# Autodesk Inventor assembly: MotorJaguarBoard
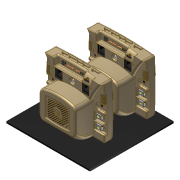
[picture p0: Inventor's stored thumbnail of the model, 180x180]
Saved by Autodesk Inventor 2012 (Build 160160000, 160)
## iProperties
Created: 2012-01-21
Part Number: MotorJaguarBoard
Document SubType Name: Assembly
Designer: JesseK
Author: JesseK
## Documents named in this file (3)
- Z:\UserData\Documents\Inventor\team1885frc\Robot2012\Electronics Board\MotorJaguarBoard.iam
- Z:\UserData\Documents\Inventor\team1885frc\Robot2012\Electronics Board\MotorJaguarBoard.ipt
- Z:\UserData\Documents\Inventor\team1885frc\Electronics\Jag\Jag.iam
## Components (3 placed, 2 different names)
1. MotorJaguarBoard:1 — Mate:1, Mate:2, Flush:1
2. Jag:1 [sub-assembly] — Mate:2, Flush:2
3. Jag:2 [sub-assembly] — Mate:1, Flush:1, Flush:2
## Relationships (4: Mate 2, Flush 2)
- Mate:1: MotorJaguarBoard:1 ↔ Jag:2
- Mate:2: MotorJaguarBoard:1 ↔ Jag:1
- Flush:1 (6.35 mm): MotorJaguarBoard:1 ↔ Jag:2
- Flush:2 (76.2 mm): Jag:1 ↔ Jag:2
